# Autodesk Inventor assembly: 2060
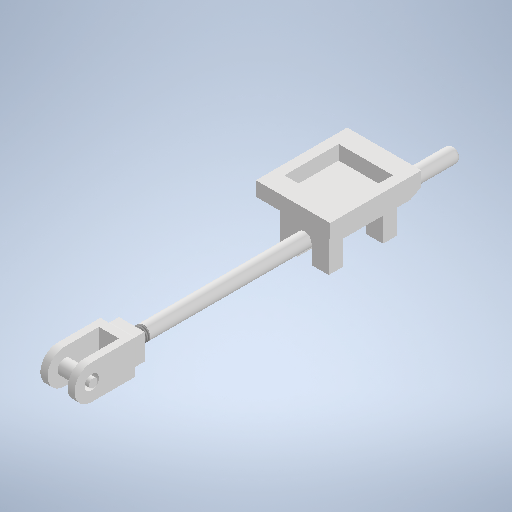
[picture p0: Inventor's stored thumbnail of the model, 512x512]
Saved by Autodesk Inventor 2025 (Build 290162010, 162A)
## iProperties
Created: 2024-05-30
Part Number: 2060
Document SubType Name: Assembly
Designer: Fabri
Author: Fabri
## Documents named in this file (5)
- C:\Users\Fabri\Documents\Inventor\Paddle\2060.iam
- C:\Users\Fabri\Documents\Inventor\Paddle\2062.ipt
- C:\Users\Fabri\Documents\Inventor\Paddle\2601.ipt
- C:\Users\Fabri\Documents\Inventor\Paddle\2063.ipt
- C:\Users\Fabri\Documents\Inventor\Paddle\2063_1.ipt
## Components (4 placed, 4 different names)
1. 2062:1 — Mate:1, Insert:1, Mate:2, Insert:2
2. 2601:1 — Mate:2, Insert:2, Angle:1
3. 2063:1 — Mate:1, Insert:1, Angle:1, Mate:3, Insert:3
4. 2063_1:1 — Mate:3, Insert:3
## Relationships (7: Mate 3, Insert 3, Angle 1)
- Mate:1: 2062:1 ↔ 2063:1
- Insert:1 (-8 mm): 2062:1 ↔ 2063:1
- Mate:2: 2062:1 ↔ 2601:1
- Insert:2 (-51.057 mm): 2062:1 ↔ 2601:1
- Angle:1 (0 deg): 2601:1 ↔ 2063:1
- Mate:3: 2063:1 ↔ 2063_1:1
- Insert:3: 2063:1 ↔ 2063_1:1
